# Autodesk Inventor assembly: Assembly_XYZ_Stage_Micrometer_ontop_lightsheet
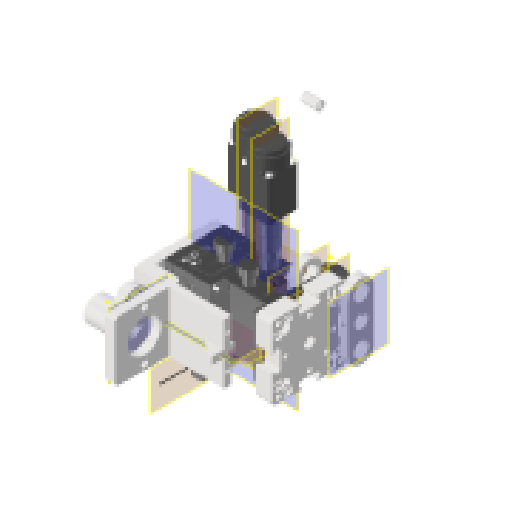
[picture p0: Inventor's stored thumbnail of the model, 512x512]
Saved by Autodesk Inventor 2025.1 (Build 291241020, 241B)
## iProperties
Created: 2023-02-07
Part Number: Assembly_XYZ_Stage_Micrometer_ontop_lightsheet
Document SubType Name: Assembly
Designer: diederichbenedict
Author: diederichbenedict
## Documents named in this file (11)
- C:\Users\diederichbenedict\Dropbox\Dokumente\Promotion\PROJECTS\openUC2-CAD\INVENTOR\Assembly_XYZ_Stage_Micrometer_ontop_lightsheet.iam
- C:\Users\diederichbenedict\Dropbox\Dokumente\Promotion\PROJECTS\openUC2-CAD\INVENTOR\00_XYZstage_micro_LT-4047-S1.ipt
- C:\Users\diederichbenedict\Dropbox\Dokumente\Promotion\PROJECTS\openUC2-CAD\INVENTOR\00_Joy-IT-B20SHD4353_NEMA8_captive.ipt
- C:\Users\diederichbenedict\Dropbox\Dokumente\Promotion\PROJECTS\openUC2-CAD\INVENTOR\40_XYZstage_micrometer_motorized_nema8_cube_ontop.ipt
- C:\Users\diederichbenedict\Dropbox\Dokumente\Promotion\PROJECTS\openUC2-CAD\INVENTOR\40_XYZstage_micrometer_motorized_nema8_lightsheet_samplemount_ontop.ipt
- C:\Users\diederichbenedict\Dropbox\Dokumente\Promotion\PROJECTS\openUC2-CAD\INVENTOR\20_Cube_Insert_Lightsheet_syringe_Rotating_hollomotor_nut_v0.ipt
- C:\Users\diederichbenedict\Dropbox\Dokumente\Promotion\PROJECTS\openUC2-CAD\INVENTOR\40_XYZstage_micrometer_motorized_nema8_zadapter_m2.5nut.ipt
- C:\Users\diederichbenedict\Dropbox\Dokumente\Promotion\PROJECTS\openUC2-CAD\INVENTOR\40_XYZstage_micrometer_motorized_nema8_samplemount_lightsheet_screwed.ipt
- C:\Users\diederichbenedict\Dropbox\Dokumente\Promotion\PROJECTS\openUC2-CAD\INVENTOR\40_XYZstage_micrometer_motorized_nema8_samplemount_lightsheet_syringemount_screwed.ipt
- C:\Users\diederichbenedict\Dropbox\Dokumente\Promotion\PROJECTS\openUC2-CAD\INVENTOR\40_XYZstage_micrometer_motorized_nema8_samplemount_lightsheet_feptube25_screwed.ipt
- C:\Users\diederichbenedict\Dropbox\Dokumente\Promotion\PROJECTS\openUC2-CAD\INVENTOR\40_XYZstage_micrometer_motorized_nema8_samplemount_lightsheet_feptube50_screwed.ipt
## Components (12 placed, 10 different names)
1. 00_XYZstage_micro_LT-4047-S1:1 — Flush:1, Flush:2, Flush:3, Flush:4, Insert:6, Angle:1
2. 00_Joy-IT-B20SHD4353_NEMA8_captive:2
3. 00_Joy-IT-B20SHD4353_NEMA8_captive:1
4. 00_Joy-IT-B20SHD4353_NEMA8_captive:3
5. 40_XYZstage_micrometer_motorized_nema8_cube_ontop:1 — Flush:1, Flush:2
6. 40_XYZstage_micrometer_motorized_nema8_lightsheet_samplemount_ontop:1 — Flush:3, Flush:4
7. 20_Cube_Insert_Lightsheet_syringe_Rotating_hollomotor_nut_v0:1
8. 40_XYZstage_micrometer_motorized_nema8_zadapter_m2.5nut:1
9. 40_XYZstage_micrometer_motorized_nema8_samplemount_lightsheet_screwed:1 — Insert:6, Angle:1, Insert:7, Angle:2
10. 40_XYZstage_micrometer_motorized_nema8_samplemount_lightsheet_feptube50_screwed:1 — Insert:7, Angle:2
11. 40_XYZstage_micrometer_motorized_nema8_samplemount_lightsheet_syringemount_screwed:1
12. 40_XYZstage_micrometer_motorized_nema8_samplemount_lightsheet_feptube25_screwed:1
## Relationships (11: Insert 5, Flush 4, Angle 2)
- [Insert]: 00_XYZstage_micro_LT-4047-S1:1 ↔ 00_Joy-IT-B20SHD4353_NEMA8_captive:1
- [Insert]: 00_XYZstage_micro_LT-4047-S1:1 ↔ 00_Joy-IT-B20SHD4353_NEMA8_captive:2
- [Insert]: 00_XYZstage_micro_LT-4047-S1:1 ↔ 00_Joy-IT-B20SHD4353_NEMA8_captive:3
- Flush:1: 00_XYZstage_micro_LT-4047-S1:1 ↔ 40_XYZstage_micrometer_motorized_nema8_cube_ontop:1
- Flush:2: 00_XYZstage_micro_LT-4047-S1:1 ↔ 40_XYZstage_micrometer_motorized_nema8_cube_ontop:1
- Flush:3: 00_XYZstage_micro_LT-4047-S1:1 ↔ 40_XYZstage_micrometer_motorized_nema8_lightsheet_samplemount_ontop:1
- Flush:4: 00_XYZstage_micro_LT-4047-S1:1 ↔ 40_XYZstage_micrometer_motorized_nema8_lightsheet_samplemount_ontop:1
- Insert:6: 00_XYZstage_micro_LT-4047-S1:1 ↔ 40_XYZstage_micrometer_motorized_nema8_samplemount_lightsheet_screwed:1
- Angle:1 (180 deg): 00_XYZstage_micro_LT-4047-S1:1 ↔ 40_XYZstage_micrometer_motorized_nema8_samplemount_lightsheet_screwed:1
- Insert:7: 40_XYZstage_micrometer_motorized_nema8_samplemount_lightsheet_screwed:1 ↔ 40_XYZstage_micrometer_motorized_nema8_samplemount_lightsheet_feptube50_screwed:1
- Angle:2 (-90 deg): 40_XYZstage_micrometer_motorized_nema8_samplemount_lightsheet_screwed:1 ↔ 40_XYZstage_micrometer_motorized_nema8_samplemount_lightsheet_feptube50_screwed:1
